# Autodesk Inventor assembly: Single Acting Piston
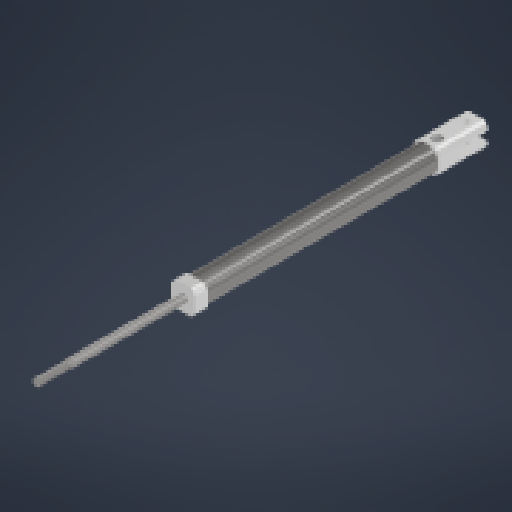
[picture p0: Inventor's stored thumbnail of the model, 512x512]
Saved by Autodesk Inventor 2024 (Build 280153000, 153)
## iProperties
Created: 2022-09-23
Part Number: Single Acting Piston
Document SubType Name: Assembly
Designer: maxxw
Mass: 12.2112 g
Surface Area: 100.21 cm^2
Volume: 12.2112 cm^3
Author: maxxw
## Documents named in this file (3)
- \\Mac\Home\Desktop\code\1899V-VRC\Cad\Motion\Pneumatics\Single Acting Piston.iam
- \\Mac\Home\Desktop\code\1899V-VRC\Cad\Motion\Pneumatics\Reference Parts\Pistons\Single Acting Piston Rod.ipt
- \\Mac\Home\Desktop\code\1899V-VRC\Cad\Motion\Pneumatics\Reference Parts\Pistons\Single Acting Piston Body.ipt
## Components (2 placed, 2 different names)
1. Single Acting Piston Rod:1 — Mate:1, Mate:2
2. Single Acting Piston Body:1 — Mate:1, Mate:2
## Relationships (2: Mate 2)
- Mate:1: Single Acting Piston Rod:1 ↔ Single Acting Piston Body:1
- Mate:2: Single Acting Piston Rod:1 ↔ Single Acting Piston Body:1
